# Autodesk Inventor assembly: Final Assembly BC
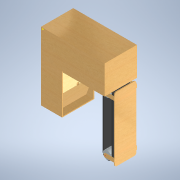
[picture p0: Inventor's stored thumbnail of the model, 180x180]
Saved by Autodesk Inventor 2022.2 (Build 262287000, 287)
## iProperties
Created: 2022-02-28
Part Number: Final Assembly BC
Document SubType Name: Assembly
Designer: PRASHANTH
Author: PRASHANTH
## Documents named in this file (4)
- E:\BME\Autodesk Sample\Engg Exploration\Final Assembly BC.iam
- E:\BME\Autodesk Sample\Engg Exploration\Subsystem1-Conveyor Belt\Assembly of Conveyor Belt.iam
- E:\BME\Autodesk Sample\Engg Exploration\Subsystem2-Storage Unit\container unit.ipt
- E:\BME\Autodesk Sample\Engg Exploration\Subsystem3-Button Unit\Assembly3.iam
## Components (3 placed, 3 different names)
1. Assembly of Conveyor Belt:1 [sub-assembly] — Flush:3, Flush:4, Mate:2
2. container unit:1 — Mate:1, Flush:1, Flush:2, Flush:5
3. Assembly3:1 [sub-assembly] — Mate:1, Flush:1, Flush:2, Flush:3, Flush:4, Mate:2, Flush:5
## Relationships (7: Flush 5, Mate 2)
- Mate:1: container unit:1 ↔ Assembly3:1
- Flush:1: container unit:1 ↔ Assembly3:1
- Flush:2: container unit:1 ↔ Assembly3:1
- Flush:3: Assembly of Conveyor Belt:1 ↔ Assembly3:1
- Flush:4: Assembly of Conveyor Belt:1 ↔ Assembly3:1
- Mate:2 (10 mm): Assembly of Conveyor Belt:1 ↔ Assembly3:1
- Flush:5: container unit:1 ↔ Assembly3:1
